# Autodesk Inventor assembly: Built Platform (metal) + Clamp Ring
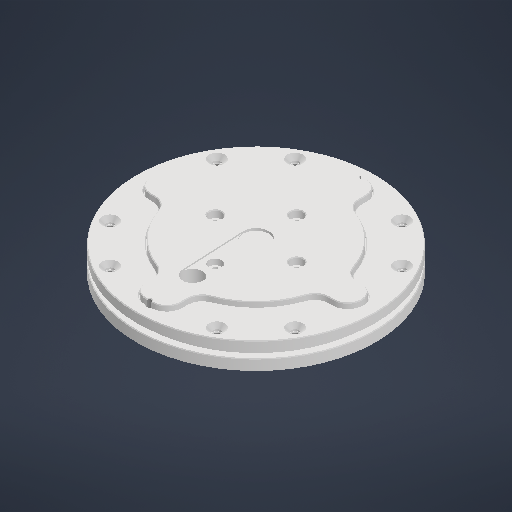
[picture p0: Inventor's stored thumbnail of the model, 512x512]
Saved by Autodesk Inventor 2025 (Build 290162000, 162)
## iProperties
Created: 2024-12-13
Part Number: Built Platform (metal) + Clamp Ring
Document SubType Name: Assembly
Designer: mayhe
Author: mayhe
## Documents named in this file (3)
- C:\Users\mayhe\OneDrive\Documents\GitHub\In-situ-monitoring-of-powder-bed-fusion-additive-manufacturing\system_development\Orichalcum\v0.2\Hardware_design\pzt-parts\Assemblies\Built Platform (metal) + Clamp Ring.iam
- C:\Users\mayhe\OneDrive\Documents\GitHub\In-situ-monitoring-of-powder-bed-fusion-additive-manufacturing\system_development\Orichalcum\v0.2\Hardware_design\pzt-parts\Build Platform\Metal\Build Plateform one Indents (metal).ipt
- C:\Users\mayhe\OneDrive\Documents\GitHub\In-situ-monitoring-of-powder-bed-fusion-additive-manufacturing\system_development\Orichalcum\v0.2\Hardware_design\pzt-parts\Build Platform\Clamp Ring.ipt
## Components (2 placed, 2 different names)
1. Build Plateform one Indents (metal):1 — Rotational:1
2. Clamp Ring:1 — Rotational:1
## Relationships (1: RevoluteJoint 1)
- Rotational:1 [RevoluteJoint]: Build Plateform one Indents (metal):1 ↔ Clamp Ring:1
